# Autodesk Inventor assembly: 20X20lift
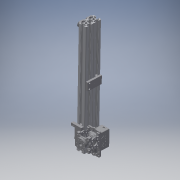
[picture p0: Inventor's stored thumbnail of the model, 180x180]
Saved by Autodesk Inventor 2017 (Build 210142000, 142)
## iProperties
Created: 2017-12-15
Part Number: 20X20lift
Document SubType Name: Assembly
Designer: User
Author: User
## Documents named in this file (12)
- C:\Robotics\CAD\2017-18_CAD\20X20lift.iam
- C:\Robotics\CAD\2017-18_CAD\Prototypes\Sliderfor2020.ipt
- C:\Robotics\CAD\COTSParts\Bosch Extrusion\Bosch 20x20 11.ipt
- C:\Robotics\CAD\2017-18_CAD\Prototypes\ServosSlideforLift.ipt
- C:\Robotics\CAD\2017-18_CAD\ShoulderScrewHolderSlide.ipt
- C:\Robotics\CAD\COTSParts\Rev\REV-41-1097.ipt
- C:\Robotics\CAD\COTSParts\Actobotics\637 parts\637112\575112.ipt
- C:\Robotics\CAD\COTSParts\Actobotics\637 parts\637112\545420.ipt
- C:\Robotics\CAD\COTSParts\Actobotics\637 parts\637112\535118 assembly.ipt
- C:\Robotics\CAD\COTSParts\Actobotics\637 parts\637112\525123.ipt
- C:\Robotics\CAD\COTSParts\Fasteners\90265A112_18-8 STAINLESS STEEL SHOULDER SCREW.ipt
- C:\Robotics\CAD\COTSParts\Rev\PulleysREV-41-1368.ipt
## Components (19 placed, 11 different names)
1. Sliderfor2020:2 — Mate:10, Mate:11, Insert:20
2. Sliderfor2020:3 — Mate:5, Mate:6, Mate:8, Mate:9
3. Bosch 20x20 11:1 — Mate:5, Mate:6, Mate:11, Flush:5, Mate:25, Mate:26, Flush:8
4. Bosch 20x20 11:2 — Mate:8, Mate:9, Mate:10, Flush:5, Mate:23, Flush:7, Mate:24, Mate:27, Mate:28, Flush:9
5. ServosSlideforLift:1 — Mate:27, Mate:28, Insert:26, Insert:27
6. ShoulderScrewHolderSlide:1 — Mate:25, Mate:26, Flush:8, Insert:21
7. ShoulderScrewHolderSlide:2 — Mate:23, Flush:7, Mate:24, Insert:22
8. REV-41-1097:1 — Insert:11, Angle:1, Insert:12
9. 575112:1 — Insert:11, Angle:1, Insert:17, Angle:2, Flush:9
10. 545420:1 — Insert:13, Insert:14, Insert:17, Angle:2, Insert:26, Insert:27
11. 525123:1 — Insert:12
12. 545420:2 — Insert:15, Insert:16
13. 535118 assembly:1 — Insert:13, Insert:14, Insert:15, Insert:16
14. 90265A112_18-8 STAINLESS STEEL SHOULDER SCREW:1 — Insert:20, Insert:25
15. 90265A112_18-8 STAINLESS STEEL SHOULDER SCREW:2 — Insert:22, Insert:24
16. 90265A112_18-8 STAINLESS STEEL SHOULDER SCREW:3 — Insert:21, Insert:23
17. PulleysREV-41-1368:1 — Insert:23
18. PulleysREV-41-1368:2 — Insert:24
19. PulleysREV-41-1368:3 — Insert:25
## Relationships (33: Insert 15, Mate 12, Flush 4, Angle 2)
- Mate:5: Sliderfor2020:3 ↔ Bosch 20x20 11:1
- Mate:6: Sliderfor2020:3 ↔ Bosch 20x20 11:1
- Mate:8: Sliderfor2020:3 ↔ Bosch 20x20 11:2
- Mate:9: Sliderfor2020:3 ↔ Bosch 20x20 11:2
- Mate:10: Sliderfor2020:2 ↔ Bosch 20x20 11:2
- Mate:11: Sliderfor2020:2 ↔ Bosch 20x20 11:1
- Flush:5: Bosch 20x20 11:1 ↔ Bosch 20x20 11:2
- Mate:23: Bosch 20x20 11:2 ↔ ShoulderScrewHolderSlide:2
- Flush:7: Bosch 20x20 11:2 ↔ ShoulderScrewHolderSlide:2
- Mate:24 (-10 mm): Bosch 20x20 11:2 ↔ ShoulderScrewHolderSlide:2
- Mate:25: Bosch 20x20 11:1 ↔ ShoulderScrewHolderSlide:1
- Mate:26 (-10 mm): Bosch 20x20 11:1 ↔ ShoulderScrewHolderSlide:1
- Flush:8: Bosch 20x20 11:1 ↔ ShoulderScrewHolderSlide:1
- Insert:11 (-2.667 mm): REV-41-1097:1 ↔ 575112:1
- Angle:1 (0 deg): REV-41-1097:1 ↔ 575112:1
- Insert:12 (1.905 mm): REV-41-1097:1 ↔ 525123:1
- Insert:13: 545420:1 ↔ 535118 assembly:1
- Insert:14: 545420:1 ↔ 535118 assembly:1
- Insert:15: 545420:2 ↔ 535118 assembly:1
- Insert:16: 545420:2 ↔ 535118 assembly:1
- Insert:17: 575112:1 ↔ 545420:1
- Angle:2 (0 deg): 575112:1 ↔ 545420:1
- Insert:20: Sliderfor2020:2 ↔ 90265A112_18-8 STAINLESS STEEL SHOULDER SCREW:1
- Insert:21: ShoulderScrewHolderSlide:1 ↔ 90265A112_18-8 STAINLESS STEEL SHOULDER SCREW:3
- Insert:22: ShoulderScrewHolderSlide:2 ↔ 90265A112_18-8 STAINLESS STEEL SHOULDER SCREW:2
- Insert:23: 90265A112_18-8 STAINLESS STEEL SHOULDER SCREW:3 ↔ PulleysREV-41-1368:1
- Insert:24: 90265A112_18-8 STAINLESS STEEL SHOULDER SCREW:2 ↔ PulleysREV-41-1368:2
- Insert:25: 90265A112_18-8 STAINLESS STEEL SHOULDER SCREW:1 ↔ PulleysREV-41-1368:3
- Mate:27: Bosch 20x20 11:2 ↔ ServosSlideforLift:1
- Mate:28: Bosch 20x20 11:2 ↔ ServosSlideforLift:1
- Insert:26: ServosSlideforLift:1 ↔ 545420:1
- Insert:27: ServosSlideforLift:1 ↔ 545420:1
- Flush:9 (1.5875 mm): Bosch 20x20 11:2 ↔ 575112:1
